# Autodesk Inventor assembly: ENSAMBLE MECANISMO DE INGRESO
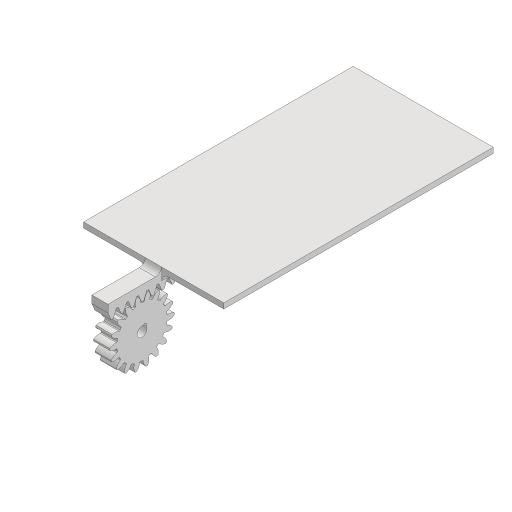
[picture p0: Inventor's stored thumbnail of the model, 512x512]
Saved by Autodesk Inventor 2024 (Build 280153000, 153)
## iProperties
Created: 2024-06-13
Part Number: ENSAMBLE MECANISMO DE INGRESO
Document SubType Name: Assembly
Designer: Jhuliams
Author: Jhuliams
## Documents named in this file (3)
- C:\Users\Jhuliams\Documents\GitHub\RECICLADOR_MODELO_3D\MECANISMO DE COMPACTADO\ENSAMBLE MECANISMO DE INGRESO.iam
- C:\Users\Jhuliams\Documents\GitHub\RECICLADOR_MODELO_3D\MECANISMO DE COMPACTADO\PINON DE TAPA PRINCIPAL.ipt
- C:\Users\Jhuliams\Documents\GitHub\RECICLADOR_MODELO_3D\MECANISMO DE COMPACTADO\TAPA PRICIPAL CON CREMALLERA.ipt
## Components (2 placed, 2 different names)
1. PINON DE TAPA PRINCIPAL:1 — Mate:1, Flush:1, Flush:2, Rotation/Translation:1
2. TAPA PRICIPAL CON CREMALLERA:1 — Flush:2, Mate:2, Rotation/Translation:1
## Relationships (6: Flush 3, Mate 2, RelateRotateTranslate 1)
- Mate:1: PINON DE TAPA PRINCIPAL:1
- Flush:1: PINON DE TAPA PRINCIPAL:1
- Flush:2: PINON DE TAPA PRINCIPAL:1 ↔ TAPA PRICIPAL CON CREMALLERA:1
- Flush:4 (27 mm)
- Mate:2 (3.75 mm): TAPA PRICIPAL CON CREMALLERA:1
- Rotation/Translation:1 [RelateRotateTranslate] (169.646 mm): PINON DE TAPA PRINCIPAL:1 ↔ TAPA PRICIPAL CON CREMALLERA:1
